# Autodesk Inventor assembly: Ensemble1
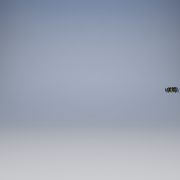
[picture p0: Inventor's stored thumbnail of the model, 180x180]
Saved by Autodesk Inventor 2019 (Build 230136000, 136)
## iProperties
Created: 2020-05-13
Part Number: Ensemble1
Material: Générique
Document SubType Name: Assembly
Designer: qrrim
Author: qrrim
## Documents named in this file (17)
- C:\Users\qrrim\OneDrive\Documents\Bachelor\S2\Projet\Plan\Ensemble1.iam
- C:\Users\qrrim\OneDrive\Documents\Bachelor\S2\Projet\Plan\Pièce élec\arduino uno.iam
- C:\Users\qrrim\OneDrive\Documents\Bachelor\S2\Projet\Plan\Barre Circulaire.ipt
- C:\Users\qrrim\OneDrive\Documents\Bachelor\S2\Projet\Plan\Cheville.ipt
- C:\Users\qrrim\OneDrive\Documents\Bachelor\S2\Projet\Plan\Jambe AR.ipt
- C:\Users\qrrim\OneDrive\Documents\Bachelor\S2\Projet\Plan\Pied.ipt
- C:\Users\qrrim\OneDrive\Documents\Bachelor\S2\Projet\Plan\Pile.ipt
- C:\Users\qrrim\OneDrive\Documents\Bachelor\S2\Projet\Plan\Pièce élec\Servo Moteur.ipt
- C:\Users\qrrim\OneDrive\Documents\Bachelor\S2\Projet\Plan\Socle P-Barre.ipt
- C:\Users\qrrim\OneDrive\Documents\Bachelor\S2\Projet\Plan\Torse.ipt
- C:\Users\qrrim\OneDrive\Documents\Bachelor\S2\Projet\Plan\Pièce élec\hc-sr04.ipt
- C:\Users\qrrim\OneDrive\Documents\Bachelor\S2\Projet\Plan\Pièce élec\Hélice SM.ipt
- C:\Users\qrrim\OneDrive\Documents\Bachelor\S2\Projet\Plan\Visse SM.ipt
- C:\Users\qrrim\OneDrive\Documents\Bachelor\S2\Projet\Plan\Pièce élec\Support.ipt
- C:\Users\qrrim\OneDrive\Documents\Bachelor\S2\Projet\Plan\Pièce élec\Gyroscope.iam
- C:\Users\qrrim\OneDrive\Documents\Bachelor\S2\Projet\Plan\Petite barre.ipt
- C:\Users\qrrim\OneDrive\Documents\Bachelor\S2\Projet\Plan\Jambe AV.ipt
## Components (34 placed, 16 different names)
1. Barre Circulaire:1 — Placage:25, Logement:44
2. Cheville:1
3. Pied:1 — Logement:43
4. Pile:1 — Placage:10, Placage:12, Placage:13
5. Servo Moteur:1 — Placage:3, Placage:4, Placage:5, Logement:3
6. Torse:1 — Placage:3, Placage:4, Placage:5, Placage:10, Placage:12, Logement:10, Placage:13, Placage:14, Placage:15, Placage:16, Placage:17, Placage:18, Placage:22, Placage:23, Logement:26, Logement:27, Logement:28, Logement:29, Logement:30, Logement:31, Logement:34, Logement:35, Logement:36
7. Cheville:2 — Logement:39, Logement:40
8. hc-sr04:2 — Logement:28, Logement:29
9. hc-sr04:3 — Logement:30, Logement:31
10. hc-sr04:4 — Logement:26, Logement:27
11. Hélice SM:1 — Logement:3, Logement:4, Logement:6, Logement:8, Logement:24, Logement:25
12. Visse SM:1 — Logement:4
13. Visse SM:2 — Logement:6
14. Visse SM:3 — Logement:8
15. Jambe AR:3 — Logement:34, Logement:40
16. Jambe AR:4 — Logement:10, Logement:42, Placage:24
17. Servo Moteur:2 — Placage:14, Placage:15, Placage:16, Logement:14
18. Hélice SM:2 — Logement:14, Logement:15, Logement:18, Logement:19, Logement:20, Logement:21
19. Visse SM:5 — Logement:19
20. Visse SM:6 — Logement:18
21. Visse SM:7 — Logement:15
22. arduino uno:1 [sub-assembly] — Placage:19, Placage:20, Placage:21
23. Support:1 — Placage:17, Placage:18, Placage:19, Placage:20, Placage:21, Placage:22
24. Gyroscope:1 [sub-assembly] — Placage:23
25. Socle P-Barre:1 — Logement:21, Logement:23
26. Socle P-Barre:2 — Logement:20, Logement:44
27. Barre Circulaire:2 — Logement:23
28. Socle P-Barre:3 — Logement:25, Logement:38
29. Socle P-Barre:4 — Logement:24, Logement:37
30. Petite barre:1 — Logement:38, Placage:24
31. Petite barre:2 — Logement:37
32. Jambe AV:1 — Logement:36, Logement:39
33. Jambe AV:2 — Logement:35, Logement:41
34. Cheville:3 — Logement:41, Logement:42, Placage:25, Logement:43
## Relationships (49: Insert 31, Mate 18)
- Placage:3 [Mate]: Servo Moteur:1 ↔ Torse:1
- Placage:4 [Mate]: Servo Moteur:1 ↔ Torse:1
- Placage:5 [Mate]: Servo Moteur:1 ↔ Torse:1
- Logement:3 [Insert]: Servo Moteur:1 ↔ Hélice SM:1
- Logement:4 [Insert]: Hélice SM:1 ↔ Visse SM:1
- Logement:6 [Insert]: Hélice SM:1 ↔ Visse SM:2
- Logement:8 [Insert]: Hélice SM:1 ↔ Visse SM:3
- Placage:10 [Mate]: Pile:1 ↔ Torse:1
- Placage:12 [Mate]: Pile:1 ↔ Torse:1
- Logement:10 [Insert]: Torse:1 ↔ Jambe AR:4
- Placage:13 [Mate]: Pile:1 ↔ Torse:1
- Placage:14 [Mate]: Torse:1 ↔ Servo Moteur:2
- Placage:15 [Mate]: Torse:1 ↔ Servo Moteur:2
- Placage:16 [Mate]: Torse:1 ↔ Servo Moteur:2
- Logement:14 [Insert]: Servo Moteur:2 ↔ Hélice SM:2
- Logement:15 [Insert]: Hélice SM:2 ↔ Visse SM:7
- Logement:18 [Insert]: Hélice SM:2 ↔ Visse SM:6
- Logement:19 [Insert]: Hélice SM:2 ↔ Visse SM:5
- Placage:17 [Mate]: Torse:1 ↔ Support:1
- Placage:18 [Mate]: Torse:1 ↔ Support:1
- Placage:19 [Mate]: arduino uno:1 ↔ Support:1
- Placage:20 [Mate]: arduino uno:1 ↔ Support:1
- Placage:21 [Mate]: arduino uno:1 ↔ Support:1
- Placage:22 [Mate]: Torse:1 ↔ Support:1
- Placage:23 [Mate]: Torse:1 ↔ Gyroscope:1
- Logement:20 [Insert]: Hélice SM:2 ↔ Socle P-Barre:2
- Logement:21 [Insert]: Hélice SM:2 ↔ Socle P-Barre:1
- Logement:23 [Insert]: Socle P-Barre:1 ↔ Barre Circulaire:2
- Logement:24 [Insert]: Hélice SM:1 ↔ Socle P-Barre:4
- Logement:25 [Insert]: Hélice SM:1 ↔ Socle P-Barre:3
- Logement:26 [Insert] (3 mm): Torse:1 ↔ hc-sr04:4
- Logement:27 [Insert] (3 mm): Torse:1 ↔ hc-sr04:4
- Logement:28 [Insert] (3 mm): Torse:1 ↔ hc-sr04:2
- Logement:29 [Insert] (3 mm): Torse:1 ↔ hc-sr04:2
- Logement:30 [Insert] (3 mm): Torse:1 ↔ hc-sr04:3
- Logement:31 [Insert] (3 mm): Torse:1 ↔ hc-sr04:3
- Logement:34 [Insert]: Torse:1 ↔ Jambe AR:3
- Logement:35 [Insert]: Torse:1 ↔ Jambe AV:2
- Logement:36 [Insert]: Torse:1 ↔ Jambe AV:1
- Logement:37 [Insert]: Socle P-Barre:4 ↔ Petite barre:2
- Logement:38 [Insert]: Socle P-Barre:3 ↔ Petite barre:1
- Logement:39 [Insert]: Cheville:2 ↔ Jambe AV:1
- Logement:40 [Insert]: Cheville:2 ↔ Jambe AR:3
- Logement:41 [Insert]: Jambe AV:2 ↔ Cheville:3
- Logement:42 [Insert]: Jambe AR:4 ↔ Cheville:3
- Placage:24 [Mate]: Jambe AR:4 ↔ Petite barre:1
- Placage:25 [Mate]: Barre Circulaire:1 ↔ Cheville:3
- Logement:43 [Insert]: Pied:1 ↔ Cheville:3
- Logement:44 [Insert]: Barre Circulaire:1 ↔ Socle P-Barre:2
